# Autodesk Inventor assembly: BC-100001-B
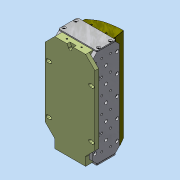
[picture p0: Inventor's stored thumbnail of the model, 180x180]
Saved by Autodesk Inventor 2016 (Build 200138000, 138)
## iProperties
Created: 2015-09-23
Part Number: BC-100001-B
Document SubType Name: Assembly
Designer: Reinaldo.Basílio
Mass: 37161.3 g
Surface Area: 6721.8 cm^2
Volume: 5243.53 cm^3
Density: 7.08707 g/cm^3
Author: Reinaldo.Basílio
## Documents named in this file (6)
- D:\ARQ\Basilio\LNLS-2\Anel\Dipolos\BC-3T\Dipolo 3T e 1T\Prototipo 1\Projeto Mecanico\BC-100001-B.iam
- D:\ARQ\Basilio\LNLS-2\Anel\Dipolos\BC-3T\Dipolo 3T e 1T\Prototipo 1\Projeto Mecanico\BC-100002.iam
- D:\ARQ\Basilio\LNLS-2\Anel\Dipolos\BC-3T\Dipolo 3T e 1T\Prototipo 1\Projeto Mecanico\BC-10004.ipt
- D:\ARQ\Basilio\LNLS-2\Anel\Dipolos\BC-3T\Dipolo 3T e 1T\Prototipo 1\Projeto Mecanico\BC-10003-B.ipt
- D:\ARQ\Basilio\LNLS-2\Anel\Dipolos\BC-3T\Dipolo 3T e 1T\Prototipo 1\Projeto Mecanico\BC-10017.ipt
- D:\ARQ\Basilio\LNLS-2\Anel\Dipolos\BC-3T\Dipolo 3T e 1T\Prototipo 1\Projeto Mecanico\BC-10024.ipt
## Components (7 placed, 5 different names)
1. BC-10003-B:1 — Flush:15, Flush:14, Mate:16, Mate:17, Flush:16, Flush:17
2. BC-100002:1 [sub-assembly] — Mate:2, Flush:7, Flush:11, Mate:17
3. BC-10004:1 — Mate:2, Flush:7, Flush:11, Insert:1, Insert:2, Insert:3, Insert:4, Flush:16, Flush:17
4. BC-10017:1 — Insert:1, Insert:2, Insert:5, Insert:8
5. BC-10017:2 — Insert:3, Insert:4, Insert:6, Insert:7
6. BC-10024:1 — Insert:5, Insert:6
7. BC-10024:2 — Insert:7, Insert:8
## Relationships (17: Insert 8, Flush 6, Mate 3)
- Mate:2: BC-100002:1 ↔ BC-10004:1
- Flush:7: BC-100002:1 ↔ BC-10004:1
- Flush:15: BC-10003-B:1
- Flush:14: BC-10003-B:1
- Flush:11: BC-100002:1 ↔ BC-10004:1
- Insert:1: BC-10004:1 ↔ BC-10017:1
- Insert:2: BC-10004:1 ↔ BC-10017:1
- Insert:3: BC-10004:1 ↔ BC-10017:2
- Insert:4: BC-10004:1 ↔ BC-10017:2
- Insert:5: BC-10017:1 ↔ BC-10024:1
- Insert:6: BC-10017:2 ↔ BC-10024:1
- Insert:7: BC-10017:2 ↔ BC-10024:2
- Insert:8: BC-10017:1 ↔ BC-10024:2
- Mate:16: BC-10003-B:1
- Mate:17: BC-10003-B:1 ↔ BC-100002:1
- Flush:16: BC-10003-B:1 ↔ BC-10004:1
- Flush:17: BC-10003-B:1 ↔ BC-10004:1
